# Autodesk Inventor assembly: Full chassis 2
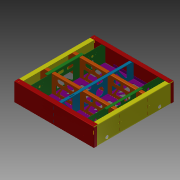
[picture p0: Inventor's stored thumbnail of the model, 180x180]
Saved by Autodesk Inventor 2015 (Build 190159000, 159)
## iProperties
Created: 2014-01-06
Part Number: Full chassis 2
Document SubType Name: Weldment
Designer: Alex
Weld Material: Welded Aluminum-6061
Mass: 8202.81 g
Surface Area: 27357.1 cm^2
Volume: 3031.7 cm^3
Density: 2.70568 g/cm^3
Author: Alex
## Documents named in this file (8)
- X:\2015 B\Full chassis-3.iam
- X:\2015 B\Front-3.ipt
- X:\2015 B\Brace-3.ipt
- X:\2015 B\InnerSide-3.ipt
- X:\2015 B\Outer_Side-3.ipt
- X:\2015 B\Base-3.ipt
- X:\2015 B\CenterBrace-3.ipt
- X:\2015 B\CenterBrace-3d.ipt
## Components (11 placed, 7 different names)
1. Brace-3:1 — Mate:15, Mate:25, Mate:37, Mate:38, Mate:39, Mate:42, Flush:7, Mate:56, Mate:57
2. Brace-3:2 — Mate:9, Mate:13, Mate:24, Mate:59, Mate:60, Flush:8
3. Front-3:1 — Mate:9, Flush:4, Mate:41, Mate:55, Mate:58
4. InnerSide-3:2 — Mate:13, Mate:15, Mate:36, Mate:49, Mate:55
5. InnerSide-3:3 — Mate:24, Mate:25, Mate:35, Mate:58
6. Front-3:2 — Mate:35, Mate:36, Flush:5, Mate:49
7. Base-3:1 — Mate:37, Mate:38, Mate:39, Mate:40, Flush:6
8. CenterBrace-3:1 — Mate:40, Flush:4, Mate:41
9. CenterBrace-3d:1 — Flush:5, Flush:6, Mate:42
10. Outer_Side-3:2 — Flush:7, Mate:56, Mate:57
11. Outer_Side-3:3 — Mate:59, Mate:60, Flush:8
## Relationships (25: Mate 20, Flush 5)
- Mate:9 (-228.6 mm): Brace-3:2 ↔ Front-3:1
- Mate:13: Brace-3:2 ↔ InnerSide-3:2
- Mate:15: Brace-3:1 ↔ InnerSide-3:2
- Mate:24: Brace-3:2 ↔ InnerSide-3:3
- Mate:25: Brace-3:1 ↔ InnerSide-3:3
- Mate:35: InnerSide-3:3 ↔ Front-3:2
- Mate:36: InnerSide-3:2 ↔ Front-3:2
- Mate:37: Brace-3:1 ↔ Base-3:1
- Mate:38: Brace-3:1 ↔ Base-3:1
- Mate:39: Brace-3:1 ↔ Base-3:1
- Mate:40: Base-3:1 ↔ CenterBrace-3:1
- Flush:4: Front-3:1 ↔ CenterBrace-3:1
- Mate:41: Front-3:1 ↔ CenterBrace-3:1
- Flush:5: Front-3:2 ↔ CenterBrace-3d:1
- Flush:6: Base-3:1 ↔ CenterBrace-3d:1
- Mate:42: Brace-3:1 ↔ CenterBrace-3d:1
- Mate:49: InnerSide-3:2 ↔ Front-3:2
- Mate:55: Front-3:1 ↔ InnerSide-3:2
- Flush:7: Brace-3:1 ↔ Outer_Side-3:2
- Mate:56: Brace-3:1 ↔ Outer_Side-3:2
- Mate:57: Brace-3:1 ↔ Outer_Side-3:2
- Mate:58: Front-3:1 ↔ InnerSide-3:3
- Mate:59: Brace-3:2 ↔ Outer_Side-3:3
- Mate:60: Brace-3:2 ↔ Outer_Side-3:3
- Flush:8: Brace-3:2 ↔ Outer_Side-3:3
